# Autodesk Inventor assembly: !drive-pod-back-left-back-right
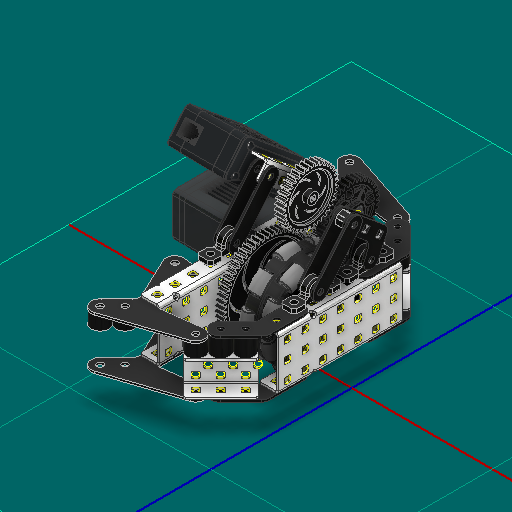
[picture p0: Inventor's stored thumbnail of the model, 512x512]
Saved by Autodesk Inventor 2025 (Build 290162000, 162)
## iProperties
Created: 2024-08-10
Part Number: !drive-pod-back-left-back-right
Document SubType Name: Assembly
Designer: averey
Author: averey
## Documents named in this file (25)
- C:\Users\avere\rbp_cad\atlas\chassis\drive-pod-back-right\!drive-pod-back-left-back-right.iam
- C:\Users\avere\rbp_cad\atlas\chassis\drive-pod-back-right\LS Pillow Bearing Block-back-left-back-right.ipt
- C:\Users\avere\rbp_cad\atlas\chassis\drive-pod-back-right\gearbox-support-gusset-back-left-back-right.ipt
- C:\Users\avere\rbp_cad\atlas\chassis\drive-pod-back-right\gearbox-gusset-back-left-back-right.ipt
- C:\Users\avere\rbp_cad\atlas\chassis\drive-pod-back-right\Bearing Flat Low Profile-back-left-back-right.ipt
- C:\Users\avere\rbp_cad\atlas\chassis\drive-pod-back-right\Alu Angle 1x1x5-back-left-back-right.ipt
- C:\Users\avere\rbp_cad\atlas\chassis\drive-pod-back-right\SteelM-StarS-back-left-back-right.iam
- C:\Users\avere\rbp_cad\atlas\chassis\drive-pod-back-right\V5 Motor (5.5W)-back-left-back-right.ipt
- C:\Users\avere\rbp_cad\atlas\chassis\drive-pod-back-right\LS 36T Gear-back-left-back-right.ipt
- C:\Users\avere\rbp_cad\atlas\chassis\drive-pod-back-right\LS 60T Gear-back-left-back-right.ipt
- C:\Users\avere\rbp_cad\atlas\chassis\drive-pod-back-right\2.75 Omni AS, No Insert-back-left-back-right.iam
- C:\Users\avere\rbp_cad\atlas\chassis\drive-pod-back-right\LS 12T Gear-back-left-back-right.ipt
- C:\Users\avere\rbp_cad\atlas\chassis\drive-pod-back-right\half_cut_36t-back-left-back-right.ipt
- C:\Users\avere\rbp_cad\atlas\chassis\drive-pod-back-right\elbow-gusset-back-left-back-right.ipt
- C:\Users\avere\rbp_cad\atlas\chassis\drive-pod-back-right\Alu C 1x2x1x3-back-left-back-right.ipt
- C:\Users\avere\rbp_cad\atlas\chassis\drive-pod-back-right\join-gusset_offset-back-left-back-right.ipt
- C:\Users\avere\rbp_cad\VEX-CAD-Inventor-1.41\Motion\Spacers\Spacer Nylon .500 OD\NSpacer Black .500 OD x .500.ipt
- C:\Users\avere\rbp_cad\VEX-CAD-Inventor-1.41\Motion\Spacers\Spacer Nylon .500 OD.ipt
- C:\Users\avere\rbp_cad\VEX-CAD-Inventor-1.41\Motion\Spacers\Spacer Nylon .500 OD\NSpacer Black .500 OD x .375.ipt
- C:\Users\avere\rbp_cad\atlas\chassis\drive-pod-back-right\Alu C 1x3x1x7-back-right.ipt
- C:\Users\avere\rbp_cad\atlas\chassis\drive-pod-back-right\Alu C 1x3x1x11-back-right.ipt
- C:\Users\avere\rbp_cad\atlas\chassis\drive-pod\custom-parts\join-gusset_offset.ipt
- C:\Users\avere\rbp_cad\VEX-CAD-Inventor-1.41\Structure\Standoff\Standoff 1.25.ipt
- C:\Users\avere\rbp_cad\VEX-CAD-Inventor-1.41\Motion\Spacers\Spacer Nylon .375 OD\NSpacer .375 OD x .125.ipt
- C:\Users\avere\rbp_cad\VEX-CAD-Inventor-1.41\Motion\Spacers\Spacer Nylon .375 OD.ipt
## Components (44 placed, 22 different names)
1. LS Pillow Bearing Block-back-left-back-right:1 — Mate:7, Insert:11, Insert:38, Mate:25
2. LS Pillow Bearing Block-back-left-back-right:2 — Insert:9, Mate:8, Mate:23, Insert:37, Mate:24
3. gearbox-support-gusset-back-left-back-right:1 — Insert:9, Insert:36, Mate:23
4. gearbox-gusset-back-left-back-right:1 — Mate:7, Mate:9, Insert:36
5. gearbox-support-gusset-back-left-back-right:2 — Mate:8
6. gearbox-gusset-back-left-back-right:2 — Insert:11, Mate:26
7. Bearing Flat Low Profile-back-left-back-right:1 — Mate:9
8. LS Pillow Bearing Block-back-left-back-right:3 — Insert:17, Insert:18, Insert:39
9. LS Pillow Bearing Block-back-left-back-right:4 — Insert:16, Insert:33, Mate:20
10. Alu Angle 1x1x5-back-left-back-right:1 — Insert:16, Mate:12, Mate:13, Insert:31, Mate:22, Insert:30, Insert:32
11. gearbox-gusset-back-left-back-right:3 — Insert:17, Mate:12, Mate:26
12. gearbox-gusset-back-left-back-right:4 — Insert:18, Mate:13
13. SteelM-StarS-back-left-back-right:1 [sub-assembly] — Insert:35, Mate:22
14. V5 Motor (5.5W)-back-left-back-right:1 — Insert:31, Mate:22
15. LS 36T Gear-back-left-back-right:1 — Insert:29
16. LS 60T Gear-back-left-back-right:1 — Mate:21, Insert:28, Insert:53
17. 2.75 Omni AS, No Insert-back-left-back-right:1 [sub-assembly] — Mate:21, Insert:28
18. LS 12T Gear-back-left-back-right:1 — Insert:29
19. half_cut_36t-back-left-back-right:1 — Insert:30
20. LS 36T Gear-back-left-back-right:2 — Insert:32
21. elbow-gusset-back-left-back-right:1 — Insert:35, Mate:25, Mate:28, Insert:45
22. Alu C 1x2x1x3-back-left-back-right:1 — Insert:35, Mate:25, Insert:41, Insert:32
23. elbow-gusset-back-left-back-right:2 — Insert:39, Insert:40
24. NSpacer Black .500 OD x .500:1 — Insert:39
25. NSpacer Black .500 OD x .500:2 — Insert:40
26. NSpacer Black .500 OD x .375:3 — Insert:41, Insert:31
27. NSpacer Black .500 OD x .375:4 — Insert:30
28. NSpacer Black .500 OD x .375:5
29. join-gusset_offset-back-left-back-right:3 — Insert:52, Mate:31, Insert:49, Insert:45
30. join-gusset_offset-back-left-back-right:4 — Mate:34, Insert:40, Insert:41, Insert:42, Insert:43
31. Alu C 1x2x1x3-back-left-back-right:2 — Insert:52, Mate:25, Insert:39, Insert:41, Insert:42
32. elbow-gusset-back-left-back-right:3 — Mate:25, Insert:39, Mate:30, Insert:47
33. NSpacer Black .500 OD x .500:6 — Insert:41
34. NSpacer Black .500 OD x .500:7 — Insert:42
35. elbow-gusset-back-left-back-right:4 — Mate:29, Insert:48, Mate:25
36. Alu C 1x3x1x7-back-right:1 — Mate:30, Mate:29, Insert:48, Insert:47, Mate:28, Insert:45, Insert:37, Mate:24, Insert:38
37. Alu C 1x3x1x11-back-right:1 — Mate:34, Insert:53, Mate:31, Insert:49, Mate:18, Mate:19, Insert:33, Mate:20, Insert:35, Mate:22, Insert:39, Insert:40
38. join-gusset_offset:1 — Insert:30, Insert:31, Mate:18
39. join-gusset_offset:2 — Insert:32, Mate:19
40. NSpacer Black .500 OD x .375:8 — Insert:41
41. NSpacer Black .500 OD x .375:9 — Insert:42
42. NSpacer Black .500 OD x .375:10 — Insert:43
43. Standoff 1.25:1 — Insert:44
44. NSpacer .375 OD x .125:1 — Insert:44, Insert:45
## Relationships (60: Insert 38, Mate 22)
- Insert:9: LS Pillow Bearing Block-back-left-back-right:2 ↔ gearbox-support-gusset-back-left-back-right:1
- Mate:7: LS Pillow Bearing Block-back-left-back-right:1 ↔ gearbox-gusset-back-left-back-right:1
- Mate:8: LS Pillow Bearing Block-back-left-back-right:2 ↔ gearbox-support-gusset-back-left-back-right:2
- Insert:11: LS Pillow Bearing Block-back-left-back-right:1 ↔ gearbox-gusset-back-left-back-right:2
- Mate:9: gearbox-gusset-back-left-back-right:1 ↔ Bearing Flat Low Profile-back-left-back-right:1
- Insert:16: LS Pillow Bearing Block-back-left-back-right:4 ↔ Alu Angle 1x1x5-back-left-back-right:1
- Insert:17 (1.5875 mm): LS Pillow Bearing Block-back-left-back-right:3 ↔ gearbox-gusset-back-left-back-right:3
- Mate:12: Alu Angle 1x1x5-back-left-back-right:1 ↔ gearbox-gusset-back-left-back-right:3
- Insert:18: LS Pillow Bearing Block-back-left-back-right:3 ↔ gearbox-gusset-back-left-back-right:4
- Mate:13: Alu Angle 1x1x5-back-left-back-right:1 ↔ gearbox-gusset-back-left-back-right:4
- Insert:31: Alu Angle 1x1x5-back-left-back-right:1 ↔ V5 Motor (5.5W)-back-left-back-right:1
- Mate:22: Alu Angle 1x1x5-back-left-back-right:1 ↔ V5 Motor (5.5W)-back-left-back-right:1
- Mate:21: LS 60T Gear-back-left-back-right:1 ↔ 2.75 Omni AS, No Insert-back-left-back-right:1
- Insert:28 (19.05 mm): LS 60T Gear-back-left-back-right:1 ↔ 2.75 Omni AS, No Insert-back-left-back-right:1
- Insert:29: LS 36T Gear-back-left-back-right:1 ↔ LS 12T Gear-back-left-back-right:1
- Insert:30 (11.5094 mm): Alu Angle 1x1x5-back-left-back-right:1 ↔ half_cut_36t-back-left-back-right:1
- Insert:32 (12.7 mm): Alu Angle 1x1x5-back-left-back-right:1 ↔ LS 36T Gear-back-left-back-right:2
- Insert:35: elbow-gusset-back-left-back-right:1 ↔ Alu C 1x2x1x3-back-left-back-right:1
- Mate:25: elbow-gusset-back-left-back-right:1 ↔ Alu C 1x2x1x3-back-left-back-right:1
- Insert:39: elbow-gusset-back-left-back-right:2 ↔ NSpacer Black .500 OD x .500:1
- Insert:40: elbow-gusset-back-left-back-right:2 ↔ NSpacer Black .500 OD x .500:2
- Insert:41: Alu C 1x2x1x3-back-left-back-right:1 ↔ NSpacer Black .500 OD x .375:3
- Insert:52: join-gusset_offset-back-left-back-right:3 ↔ Alu C 1x2x1x3-back-left-back-right:2
- Mate:25: Alu C 1x2x1x3-back-left-back-right:2 ↔ elbow-gusset-back-left-back-right:3
- Insert:39: Alu C 1x2x1x3-back-left-back-right:2 ↔ elbow-gusset-back-left-back-right:3
- Insert:41: Alu C 1x2x1x3-back-left-back-right:2 ↔ NSpacer Black .500 OD x .500:6
- Insert:42: Alu C 1x2x1x3-back-left-back-right:2 ↔ NSpacer Black .500 OD x .500:7
- Mate:30: elbow-gusset-back-left-back-right:3 ↔ Alu C 1x3x1x7-back-right:1
- Mate:29: elbow-gusset-back-left-back-right:4 ↔ Alu C 1x3x1x7-back-right:1
- Insert:48: elbow-gusset-back-left-back-right:4 ↔ Alu C 1x3x1x7-back-right:1
- Insert:47: elbow-gusset-back-left-back-right:3 ↔ Alu C 1x3x1x7-back-right:1
- Mate:28: elbow-gusset-back-left-back-right:1 ↔ Alu C 1x3x1x7-back-right:1
- Insert:45: elbow-gusset-back-left-back-right:1 ↔ Alu C 1x3x1x7-back-right:1
- Mate:34: join-gusset_offset-back-left-back-right:4 ↔ Alu C 1x3x1x11-back-right:1
- Insert:53 (0.3969 mm): LS 60T Gear-back-left-back-right:1 ↔ Alu C 1x3x1x11-back-right:1
- Mate:31: join-gusset_offset-back-left-back-right:3 ↔ Alu C 1x3x1x11-back-right:1
- Insert:49: join-gusset_offset-back-left-back-right:3 ↔ Alu C 1x3x1x11-back-right:1
- Insert:30: NSpacer Black .500 OD x .375:4 ↔ join-gusset_offset:1
- Insert:31: NSpacer Black .500 OD x .375:3 ↔ join-gusset_offset:1
- Mate:18: Alu C 1x3x1x11-back-right:1 ↔ join-gusset_offset:1
- Insert:32: Alu C 1x2x1x3-back-left-back-right:1 ↔ join-gusset_offset:2
- Mate:19: Alu C 1x3x1x11-back-right:1 ↔ join-gusset_offset:2
- Insert:33: LS Pillow Bearing Block-back-left-back-right:4 ↔ Alu C 1x3x1x11-back-right:1
- Mate:20: LS Pillow Bearing Block-back-left-back-right:4 ↔ Alu C 1x3x1x11-back-right:1
- Insert:35: SteelM-StarS-back-left-back-right:1 ↔ Alu C 1x3x1x11-back-right:1
- Mate:22: SteelM-StarS-back-left-back-right:1 ↔ Alu C 1x3x1x11-back-right:1
- Insert:36: gearbox-support-gusset-back-left-back-right:1 ↔ gearbox-gusset-back-left-back-right:1
- Mate:23: LS Pillow Bearing Block-back-left-back-right:2 ↔ gearbox-support-gusset-back-left-back-right:1
- Insert:37 (4.7625 mm): LS Pillow Bearing Block-back-left-back-right:2 ↔ Alu C 1x3x1x7-back-right:1
- Mate:24: LS Pillow Bearing Block-back-left-back-right:2 ↔ Alu C 1x3x1x7-back-right:1
- Insert:38 (3.175 mm): LS Pillow Bearing Block-back-left-back-right:1 ↔ Alu C 1x3x1x7-back-right:1
- Mate:25: LS Pillow Bearing Block-back-left-back-right:1 ↔ elbow-gusset-back-left-back-right:4
- Mate:26: gearbox-gusset-back-left-back-right:2 ↔ gearbox-gusset-back-left-back-right:3
- Insert:39 (3.175 mm): LS Pillow Bearing Block-back-left-back-right:3 ↔ Alu C 1x3x1x11-back-right:1
- Insert:40: join-gusset_offset-back-left-back-right:4 ↔ Alu C 1x3x1x11-back-right:1
- Insert:41: join-gusset_offset-back-left-back-right:4 ↔ NSpacer Black .500 OD x .375:8
- Insert:42: join-gusset_offset-back-left-back-right:4 ↔ NSpacer Black .500 OD x .375:9
- Insert:43: join-gusset_offset-back-left-back-right:4 ↔ NSpacer Black .500 OD x .375:10
- Insert:44: Standoff 1.25:1 ↔ NSpacer .375 OD x .125:1
- Insert:45: join-gusset_offset-back-left-back-right:3 ↔ NSpacer .375 OD x .125:1
